# Autodesk Inventor assembly: Final Assembly
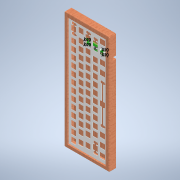
[picture p0: Inventor's stored thumbnail of the model, 180x180]
Saved by Autodesk Inventor 2022 (Build 260153000, 153)
## iProperties
Created: 2022-03-03
Part Number: Final Assembly
Document SubType Name: Assembly
Designer: Nathan Griffith
Author: Nathan Griffith
## Documents named in this file (4)
- C:\Users\Nathan Griffith\Documents\Inventor\Eric's Keyboard\Eric60percentkeyboard\Inventor\Final Assembly.iam
- C:\Users\Nathan Griffith\Documents\Inventor\Eric's Keyboard\Eric60percentkeyboard\Inventor\Case\Case Parts.ipt
- C:\Users\Nathan Griffith\Documents\Inventor\Eric's Keyboard\Eric60percentkeyboard\Inventor\Case\plate.ipt
- C:\Users\Nathan Griffith\Documents\Inventor\Eric's Keyboard\Eric60percentkeyboard\Inventor\RP pico\Raspberry Pi Pico-R3.iam
## Components (3 placed, 3 different names)
1. plate:1 — Mate:1, Mate:3, Mate:4
2. Raspberry Pi Pico-R3:1 [sub-assembly] — Flush:1, Insert:1, Insert:2
3. Case Parts:1 — Mate:1, Mate:3, Mate:4, Flush:1, Insert:1, Insert:2
## Relationships (6: Mate 3, Insert 2, Flush 1)
- Mate:1: plate:1 ↔ Case Parts:1
- Mate:3: plate:1 ↔ Case Parts:1
- Mate:4: plate:1 ↔ Case Parts:1
- Flush:1: Raspberry Pi Pico-R3:1 ↔ Case Parts:1
- Insert:1: Raspberry Pi Pico-R3:1 ↔ Case Parts:1
- Insert:2: Raspberry Pi Pico-R3:1 ↔ Case Parts:1
